# Autodesk Inventor assembly: main room, doors, corridor connected
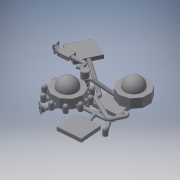
[picture p0: Inventor's stored thumbnail of the model, 180x180]
Saved by Autodesk Inventor 2017 (Build 210142000, 142)
## iProperties
Created: 2018-03-04
Part Number: main room, doors, corridor connected
Document SubType Name: Assembly
Designer: Braxton
Author: Braxton
## Documents named in this file (21)
- E:\School\Game develpment\geoscape\done solid\map\main room, doors, corridor connected.iam
- E:\School\Game develpment\geoscape\done solid\rooms\assembly\main room with double door.iam
- E:\School\Game develpment\geoscape\done solid\doors\end door\9 foot door\end door room (9).ipt
- E:\School\Game develpment\geoscape\done solid\doors\end door\9 foot door\end door assembly (closed) (9).ipt.iam
- E:\School\Game develpment\geoscape\done solid\corridors (hollow done)\corridor.ipt
- E:\School\Game develpment\geoscape\done solid\corridors (hollow done)\corridor turn.ipt
- E:\School\Game develpment\geoscape\done solid\corridors (hollow done)\Y corridor.ipt
- E:\School\Game develpment\geoscape\done solid\corridors (hollow done)\end cap.ipt
- E:\School\Game develpment\geoscape\done solid\corridors (hollow done)\curve ramp.ipt
- E:\School\Game develpment\geoscape\done solid\corridors (hollow done)\ramp top connect.ipt
- E:\School\Game develpment\geoscape\done solid\corridors (hollow done)\ramp.ipt
- E:\School\Game develpment\geoscape\done solid\corridors (hollow done)\ramp bottom connect.ipt
- E:\School\Game develpment\geoscape\done solid\rooms\dome.ipt
- E:\School\Game develpment\geoscape\done solid\rooms\assembly\assembly of dome with corridors with all doors.iam
- E:\School\Game develpment\geoscape\done solid\rooms\assembly\dome one terminal.iam
- E:\School\Game develpment\geoscape\done solid\corridors (hollow done)\X corridor.ipt
- E:\School\Game develpment\geoscape\done solid\corridors (hollow done)\ramp connect both ends.ipt
- E:\School\Game develpment\geoscape\done solid\rooms\room with 15 cubicals.ipt
- E:\School\Game develpment\geoscape\done solid\doors\end door\9 foot door\end door assembly (9).ipt.iam
- end door assembly (closed) (9).ipt
- end door assembly (9).ipt
## Components (70 placed, 18 different names)
1. corridor turn:8 — Mate:14, Flush:48, Insert:61, Insert:62
2. corridor:15 — Flush:48, Flush:49, Insert:62, Insert:63
3. corridor:16 — Flush:49, Flush:50, Insert:63, Insert:64
4. corridor:17 — Flush:50, Flush:51, Insert:64, Insert:65
5. corridor:18 — Flush:51, Flush:52, Insert:65, Insert:66
6. corridor:19 — Flush:52, Mate:15, Insert:66, Insert:67
7. end door assembly (9).ipt:1 [sub-assembly] — Mate:16, Mate:17
8. end door room (9):2 — Mate:15, Insert:67, Mate:16, Mate:17
9. ramp top connect:3 — Flush:47, Insert:57, Insert:60, Mate:11
10. ramp:8 — Flush:46, Flush:47, Insert:56, Insert:57
11. ramp:7 — Flush:45, Flush:46, Insert:55, Insert:56
12. ramp:6 — Flush:44, Flush:45, Insert:54, Insert:55
13. ramp:5 — Flush:43, Flush:44, Insert:53, Insert:54
14. ramp:4 — Flush:42, Flush:43, Insert:52, Insert:53
15. ramp bottom connect:3 — Insert:51, Flush:42, Insert:52
16. corridor turn:7 — Insert:49, Flush:41, Insert:51
17. corridor turn:6 — Insert:49, Insert:50, Flush:40, Flush:41
18. corridor:14 — Flush:36, Insert:48, Insert:50, Flush:40
19. corridor:13 — Flush:36, Flush:37, Insert:47, Insert:48
20. corridor:12 — Flush:37, Flush:38, Insert:46, Insert:47
21. corridor:11 — Flush:38, Flush:39, Insert:45, Insert:46
22. corridor:10 — Flush:39, Insert:44, Insert:45
23. corridor turn:5 — Flush:34, Insert:42, Insert:44
24. corridor:9 — Flush:33, Flush:34, Insert:41, Insert:42
25. corridor:8 — Flush:32, Flush:33, Insert:40, Insert:41
26. corridor turn:4 — Flush:31, Flush:32, Insert:39, Insert:40
27. corridor turn:3 — Flush:30, Flush:31, Insert:38, Insert:39
28. ramp top connect:2 — Insert:37, Flush:29, Flush:30, Insert:38
29. ramp bottom connect:2 — Insert:37, Flush:29, Insert:43, Flush:35
30. corridor:7 — Insert:35, Flush:28, Insert:36, Mate:10
31. corridor:6 — Insert:34, Insert:35, Flush:27, Flush:28
32. Y corridor:2 — Insert:33, Flush:26, Insert:34, Flush:27, Insert:43, Flush:35
33. corridor:5 — Insert:32, Insert:33, Flush:25, Flush:26
34. ramp connect both ends:2 — Insert:30, Flush:24, Insert:58, Mate:12
35. ramp connect both ends:1 — Insert:29, Flush:23, Insert:59, Mate:13
36. X corridor:1 — Insert:28, Insert:29, Insert:30, Flush:22, Flush:23, Flush:24, Insert:32, Flush:25
37. corridor:4 — Insert:27, Insert:28, Flush:21, Flush:22
38. corridor:3 — Insert:26, Insert:27, Flush:20, Flush:21
39. corridor turn:2 — Insert:26, Insert:31, Mate:9, Flush:20
40. end cap:3 — Insert:25, Mate:8
41. end cap:2 — Insert:24, Mate:7
42. ramp bottom connect:1 — Insert:12, Flush:9, Insert:13, Mate:6
43. ramp:3 — Insert:11, Flush:8, Insert:12, Flush:9
44. ramp:2 — Insert:10, Insert:11, Flush:7, Flush:8
45. ramp:1 — Insert:9, Insert:10, Flush:6, Flush:7
46. ramp top connect:1 — Insert:8, Mate:5, Insert:9, Flush:6
47. curve ramp:1 — Insert:7, Mate:4, Insert:8, Mate:5, Insert:14, Flush:10, Insert:24, Mate:7, Insert:25, Mate:8, Insert:31, Mate:9, Mate:14, Insert:61
48. end cap:1 — Insert:6, Flush:5
49. Y corridor:1 — Insert:5, Flush:4, Insert:6, Flush:5, Insert:7, Mate:4
50. corridor turn:1 — Insert:4, Flush:3, Insert:5, Flush:4
51. corridor:2 — Insert:3, Flush:2, Insert:4, Flush:3
52. corridor:1 — Insert:2, Insert:3, Mate:3, Flush:2
53. room with 15 cubicals:1 — Insert:58, Mate:12
54. room with 15 cubicals:2 — Insert:59, Mate:13
55. room with 15 cubicals:3 — Insert:60, Mate:11
56. assembly of dome with corridors with all doors:1 [sub-assembly] — Insert:14, Flush:10, Insert:15, Insert:16, Insert:17, Insert:18, Insert:19, Insert:20, Insert:21, Insert:22, Insert:23, Flush:11, Flush:12, Flush:13, Flush:14, Flush:15, Flush:16, Flush:17, Flush:18, Flush:19
57. main room with double door:1 [sub-assembly] — Insert:1, Flush:1, Insert:2, Mate:3
58. end door assembly (closed) (9).ipt:1 [sub-assembly] — Mate:1, Mate:2
59. end door room (9):1 — Insert:1, Flush:1, Mate:1, Mate:2
60. dome one terminal:10 [sub-assembly] — Insert:36, Mate:10
61. dome one terminal:1 [sub-assembly] — Insert:23, Flush:19
62. dome one terminal:2 [sub-assembly] — Insert:22, Flush:18
63. dome one terminal:3 [sub-assembly] — Insert:21, Flush:17
64. dome one terminal:4 [sub-assembly] — Insert:20, Flush:16
65. dome one terminal:5 [sub-assembly] — Insert:19, Flush:15
66. dome one terminal:6 [sub-assembly] — Insert:18, Flush:14
67. dome one terminal:7 [sub-assembly] — Insert:17, Flush:13
68. dome one terminal:8 [sub-assembly] — Insert:16, Flush:12
69. dome one terminal:9 [sub-assembly] — Insert:15, Flush:11
70. dome:1 — Insert:13, Mate:6
## Relationships (136: Insert 67, Flush 52, Mate 17)
- Insert:1: main room with double door:1 ↔ end door room (9):1
- Flush:1: main room with double door:1 ↔ end door room (9):1
- Mate:1: end door assembly (closed) (9).ipt:1 ↔ end door room (9):1
- Mate:2: end door assembly (closed) (9).ipt:1 ↔ end door room (9):1
- Insert:2: corridor:1 ↔ main room with double door:1
- Insert:3: corridor:2 ↔ corridor:1
- Mate:3: corridor:1 ↔ main room with double door:1
- Flush:2: corridor:2 ↔ corridor:1
- Insert:4: corridor turn:1 ↔ corridor:2
- Flush:3: corridor turn:1 ↔ corridor:2
- Insert:5: Y corridor:1 ↔ corridor turn:1
- Flush:4: Y corridor:1 ↔ corridor turn:1
- Insert:6: end cap:1 ↔ Y corridor:1
- Flush:5: end cap:1 ↔ Y corridor:1
- Insert:7: curve ramp:1 ↔ Y corridor:1
- Mate:4: curve ramp:1 ↔ Y corridor:1
- Insert:8: ramp top connect:1 ↔ curve ramp:1
- Mate:5: ramp top connect:1 ↔ curve ramp:1
- Insert:9: ramp:1 ↔ ramp top connect:1
- Insert:10: ramp:2 ↔ ramp:1
- Insert:11: ramp:3 ↔ ramp:2
- Flush:6: ramp:1 ↔ ramp top connect:1
- Flush:7: ramp:2 ↔ ramp:1
- Flush:8: ramp:3 ↔ ramp:2
- Insert:12: ramp bottom connect:1 ↔ ramp:3
- Flush:9: ramp bottom connect:1 ↔ ramp:3
- Insert:13: ramp bottom connect:1 ↔ dome:1
- Mate:6: ramp bottom connect:1 ↔ dome:1
- Insert:14: curve ramp:1 ↔ assembly of dome with corridors with all doors:1
- Flush:10: curve ramp:1 ↔ assembly of dome with corridors with all doors:1
- Insert:15: assembly of dome with corridors with all doors:1 ↔ dome one terminal:9
- Insert:16: assembly of dome with corridors with all doors:1 ↔ dome one terminal:8
- Insert:17: assembly of dome with corridors with all doors:1 ↔ dome one terminal:7
- Insert:18: assembly of dome with corridors with all doors:1 ↔ dome one terminal:6
- Insert:19: assembly of dome with corridors with all doors:1 ↔ dome one terminal:5
- Insert:20: assembly of dome with corridors with all doors:1 ↔ dome one terminal:4
- Insert:21: assembly of dome with corridors with all doors:1 ↔ dome one terminal:3
- Insert:22: assembly of dome with corridors with all doors:1 ↔ dome one terminal:2
- Insert:23: assembly of dome with corridors with all doors:1 ↔ dome one terminal:1
- Flush:11: assembly of dome with corridors with all doors:1 ↔ dome one terminal:9
- Flush:12: assembly of dome with corridors with all doors:1 ↔ dome one terminal:8
- Flush:13: assembly of dome with corridors with all doors:1 ↔ dome one terminal:7
- Flush:14: assembly of dome with corridors with all doors:1 ↔ dome one terminal:6
- Flush:15: assembly of dome with corridors with all doors:1 ↔ dome one terminal:5
- Flush:16: assembly of dome with corridors with all doors:1 ↔ dome one terminal:4
- Flush:17: assembly of dome with corridors with all doors:1 ↔ dome one terminal:3
- Flush:18: assembly of dome with corridors with all doors:1 ↔ dome one terminal:2
- Flush:19: assembly of dome with corridors with all doors:1 ↔ dome one terminal:1
- Insert:24: end cap:2 ↔ curve ramp:1
- Mate:7: end cap:2 ↔ curve ramp:1
- Insert:25: end cap:3 ↔ curve ramp:1
- Mate:8: end cap:3 ↔ curve ramp:1
- Insert:26: corridor:3 ↔ corridor turn:2
- Insert:27: corridor:4 ↔ corridor:3
- Insert:28: X corridor:1 ↔ corridor:4
- Insert:29: ramp connect both ends:1 ↔ X corridor:1
- Insert:30: ramp connect both ends:2 ↔ X corridor:1
- Insert:31: corridor turn:2 ↔ curve ramp:1
- Mate:9: corridor turn:2 ↔ curve ramp:1
- Flush:20: corridor:3 ↔ corridor turn:2
- Flush:21: corridor:4 ↔ corridor:3
- Flush:22: X corridor:1 ↔ corridor:4
- Flush:23: ramp connect both ends:1 ↔ X corridor:1
- Flush:24: ramp connect both ends:2 ↔ X corridor:1
- Insert:32: corridor:5 ↔ X corridor:1
- Insert:33: Y corridor:2 ↔ corridor:5
- Flush:25: corridor:5 ↔ X corridor:1
- Flush:26: Y corridor:2 ↔ corridor:5
- Insert:34: corridor:6 ↔ Y corridor:2
- Insert:35: corridor:7 ↔ corridor:6
- Flush:27: corridor:6 ↔ Y corridor:2
- Flush:28: corridor:7 ↔ corridor:6
- Insert:36: corridor:7 ↔ dome one terminal:10
- Mate:10: corridor:7 ↔ dome one terminal:10
- Insert:37: ramp top connect:2 ↔ ramp bottom connect:2
- Flush:29: ramp top connect:2 ↔ ramp bottom connect:2
- Flush:30: corridor turn:3 ↔ ramp top connect:2
- Flush:31: corridor turn:4 ↔ corridor turn:3
- Flush:32: corridor:8 ↔ corridor turn:4
- Flush:33: corridor:9 ↔ corridor:8
- Flush:34: corridor turn:5 ↔ corridor:9
- Insert:38: corridor turn:3 ↔ ramp top connect:2
- Insert:39: corridor turn:4 ↔ corridor turn:3
- Insert:40: corridor:8 ↔ corridor turn:4
- Insert:41: corridor:9 ↔ corridor:8
- Insert:42: corridor turn:5 ↔ corridor:9
- Insert:43: ramp bottom connect:2 ↔ Y corridor:2
- Flush:35: ramp bottom connect:2 ↔ Y corridor:2
- Flush:36: corridor:14 ↔ corridor:13
- Flush:37: corridor:13 ↔ corridor:12
- Flush:38: corridor:12 ↔ corridor:11
- Flush:39: corridor:11 ↔ corridor:10
- Insert:44: corridor:10 ↔ corridor turn:5
- Insert:45: corridor:11 ↔ corridor:10
- Insert:46: corridor:12 ↔ corridor:11
- Insert:47: corridor:13 ↔ corridor:12
- Insert:48: corridor:14 ↔ corridor:13
- Insert:49: corridor turn:7 ↔ corridor turn:6
- Insert:50: corridor turn:6 ↔ corridor:14
- Flush:40: corridor turn:6 ↔ corridor:14
- Flush:41: corridor turn:7 ↔ corridor turn:6
- Insert:51: ramp bottom connect:3 ↔ corridor turn:7
- Flush:42: ramp:4 ↔ ramp bottom connect:3
- Flush:43: ramp:5 ↔ ramp:4
- Flush:44: ramp:6 ↔ ramp:5
- Flush:45: ramp:7 ↔ ramp:6
- Flush:46: ramp:8 ↔ ramp:7
- Flush:47: ramp top connect:3 ↔ ramp:8
- Insert:52: ramp:4 ↔ ramp bottom connect:3
- Insert:53: ramp:5 ↔ ramp:4
- Insert:54: ramp:6 ↔ ramp:5
- Insert:55: ramp:7 ↔ ramp:6
- Insert:56: ramp:8 ↔ ramp:7
- Insert:57: ramp top connect:3 ↔ ramp:8
- Insert:58: ramp connect both ends:2 ↔ room with 15 cubicals:1
- Insert:59: ramp connect both ends:1 ↔ room with 15 cubicals:2
- Insert:60: ramp top connect:3 ↔ room with 15 cubicals:3
- Mate:11: ramp top connect:3 ↔ room with 15 cubicals:3
- Mate:12: ramp connect both ends:2 ↔ room with 15 cubicals:1
- Mate:13: ramp connect both ends:1 ↔ room with 15 cubicals:2
- Mate:14: corridor turn:8 ↔ curve ramp:1
- Flush:48: corridor turn:8 ↔ corridor:15
- Flush:49: corridor:15 ↔ corridor:16
- Flush:50: corridor:16 ↔ corridor:17
- Flush:51: corridor:17 ↔ corridor:18
- Flush:52: corridor:18 ↔ corridor:19
- Mate:15: corridor:19 ↔ end door room (9):2
- Insert:61: corridor turn:8 ↔ curve ramp:1
- Insert:62: corridor turn:8 ↔ corridor:15
- Insert:63: corridor:15 ↔ corridor:16
- Insert:64: corridor:16 ↔ corridor:17
- Insert:65: corridor:17 ↔ corridor:18
- Insert:66: corridor:18 ↔ corridor:19
- Insert:67: corridor:19 ↔ end door room (9):2
- Mate:16: end door assembly (9).ipt:1 ↔ end door room (9):2
- Mate:17: end door assembly (9).ipt:1 ↔ end door room (9):2
